# Autodesk Inventor assembly: Wheel Medium Omni
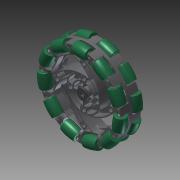
[picture p0: Inventor's stored thumbnail of the model, 180x180]
Saved by Autodesk Inventor 2015 SP1 (Build 190203100, 203)
## iProperties
Created: 2015-09-27
Part Number: Wheel Medium Omni
Document SubType Name: Assembly
Designer: Christopher
Author: Christopher
## Documents named in this file (3)
- F:\VEX CAD Library\Motion\Wheel Medium Omni.iam
- F:\VEX CAD Library\Motion\Insert HS Metal.ipt
- F:\VEX CAD Library\Motion\Wheel Medium Omni.ipt
## Components (3 placed, 2 different names)
1. Insert HS Metal:1 — Mate:1, Mate:2, Angle:1
2. Wheel Medium Omni:1 — Mate:1, Mate:2, Angle:1, Angle:2, Mate:3, Mate:4, Mate:5, Mate:6
3. Insert HS Metal:2 — Angle:2, Mate:3, Mate:4
## Relationships (8: Mate 6, Angle 2)
- Mate:1: Insert HS Metal:1 ↔ Wheel Medium Omni:1
- Mate:2: Insert HS Metal:1 ↔ Wheel Medium Omni:1
- Angle:1 (0 deg): Insert HS Metal:1 ↔ Wheel Medium Omni:1
- Angle:2 (0 deg): Wheel Medium Omni:1 ↔ Insert HS Metal:2
- Mate:3: Wheel Medium Omni:1 ↔ Insert HS Metal:2
- Mate:4: Wheel Medium Omni:1 ↔ Insert HS Metal:2
- Mate:5: Wheel Medium Omni:1
- Mate:6: Wheel Medium Omni:1
